# Autodesk Inventor assembly: RPLIDAR A1M8 (iges)
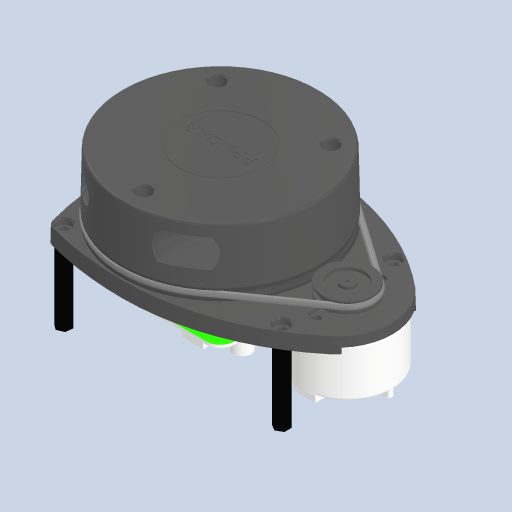
[picture p0: Inventor's stored thumbnail of the model, 512x512]
Saved by Autodesk Inventor 2024 (Build 280153000, 153)
## iProperties
Created: 2021-06-01
Part Number: RPLIDAR A1M8 (iges)
Description: SolidWorks IGES file using analytic representation for surfaces
Document SubType Name: Assembly
Designer: Greg
Sending System: SolidWorks 2020
Preprocessor: SolidWorks 2020
Minimum Resolution: 0.0
Sending System Product ID: ϞП-RPLIDAR-1.5 - R6
Receiving System Product ID: ϞП-RPLIDAR-1.5 - R6
Sent Units: Millimeter
Translation Standard: IGES 5.3
Model Creation Time: 2021-06-01
Author: WangYC
## Documents named in this file (23)
- C:\Users\Greg\Documents\Inventor\Capstone\RPLIDAR A1M8\RPLIDAR A1M8.iam
- C:\Users\Greg\Documents\Inventor\Capstone\RPLIDAR A1M8\6807.ipt
- C:\Users\Greg\Documents\Inventor\Capstone\RPLIDAR A1M8\1.25 4pin.ipt
- C:\Users\Greg\Documents\Inventor\Capstone\RPLIDAR A1M8\1.25 3pin.ipt
- C:\Users\Greg\Documents\Inventor\Capstone\RPLIDAR A1M8\1.25 2pin-2.ipt
- C:\Users\Greg\Documents\Inventor\Capstone\RPLIDAR A1M8\1.25 2pin-1.ipt
- C:\Users\Greg\Documents\Inventor\Capstone\RPLIDAR A1M8\short metal version-2.ipt
- C:\Users\Greg\Documents\Inventor\Capstone\RPLIDAR A1M8\Standoff.ipt
- C:\Users\Greg\Documents\Inventor\Capstone\RPLIDAR A1M8\Platform.ipt
- C:\Users\Greg\Documents\Inventor\Capstone\RPLIDAR A1M8\Belt-RPLIDAR-1.5 - R6.ipt
- C:\Users\Greg\Documents\Inventor\Capstone\RPLIDAR A1M8\Turntable.ipt
- C:\Users\Greg\Documents\Inventor\Capstone\RPLIDAR A1M8\InnerPCB.ipt
- C:\Users\Greg\Documents\Inventor\Capstone\RPLIDAR A1M8\Small Hole.ipt
- C:\Users\Greg\Documents\Inventor\Capstone\RPLIDAR A1M8\Big Hole.ipt
- C:\Users\Greg\Documents\Inventor\Capstone\RPLIDAR A1M8\Dome.ipt
- C:\Users\Greg\Documents\Inventor\Capstone\RPLIDAR A1M8\Motor.ipt
- C:\Users\Greg\Documents\Inventor\Capstone\RPLIDAR A1M8\Pulley.ipt
- C:\Users\Greg\Documents\Inventor\Capstone\RPLIDAR A1M8\Reciever.ipt
- C:\Users\Greg\Documents\Inventor\Capstone\RPLIDAR A1M8\Slip Head.ipt
- C:\Users\Greg\Documents\Inventor\Capstone\RPLIDAR A1M8\PCB.ipt
- C:\Users\Greg\Documents\Inventor\Capstone\RPLIDAR A1M8\Inner Standoff.ipt
- C:\Users\Greg\Documents\Inventor\Capstone\RPLIDAR A1M8\Emitter.ipt
- C:\Users\Greg\Documents\Inventor\Capstone\RPLIDAR A1M8\Back Plate.ipt
## Components (27 placed, 22 different names)
1. Platform — Mate:1, Mate:2, Insert:1, Insert:2, Insert:3
2. 6807
3. Turntable
4. Inner PCB
5. Small Hole
6. Big Hole
7. Dome
8. Motor
9. Pulley
10. Receiver
11. Slip Head
12. Belt-RPLIDAR-1.5 - R6
13. PCB
14. 1.25 4pin
15. 1.25 3pin
16. 1.25 2pin-2
17. 1.25 2pin-1
18. Inner Standoff
19. Inner Standoff:2
20. Inner Standoff:3
21. short metal version-2
22. Emitter
23. Back Plate
24. Standoff:1 — Mate:1, Mate:2
25. Standoff:2 — Insert:1
26. Standoff:3 — Insert:2
27. Standoff:4 — Insert:3
## Relationships (5: Insert 3, Mate 2)
- Mate:1: Platform ↔ Standoff:1
- Mate:2: Platform ↔ Standoff:1
- Insert:1: Platform ↔ Standoff:2
- Insert:2: Platform ↔ Standoff:3
- Insert:3: Platform ↔ Standoff:4
